# Autodesk Inventor assembly: GFRP_T2_06
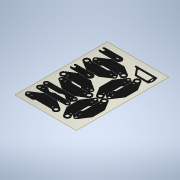
[picture p0: Inventor's stored thumbnail of the model, 180x180]
Saved by Autodesk Inventor 2020 (Build 240168000, 168)
## iProperties
Created: 2021-08-27
Part Number: GFRP_T2_06
Document SubType Name: Assembly
Designer: Masato
Author: Masato
## Documents named in this file (6)
- C:\Users\naoki\Documents\Inventor\CitBrains\git_clone\SUSTAINA_ver1_0\A_T2_175\SUSTAINA-OP\Cam\GFRP_T2_06.iam
- C:\Users\naoki\Documents\Inventor\CitBrains\git_clone\SUSTAINA_ver1_0\A_T2_175\SUSTAINA-OP\Cam\DisposableBoard.ipt
- C:\Users\naoki\Documents\Inventor\CitBrains\git_clone\SUSTAINA_ver1_0\A_T2_175\SUSTAINA-OP\LowerBody\Link\BackLink_frame.ipt
- C:\Users\naoki\Documents\Inventor\CitBrains\git_clone\SUSTAINA_ver1_0\A_T2_175\SUSTAINA-OP\LowerBody\Link\FrontLink_frame.ipt
- C:\Users\naoki\Documents\Inventor\CitBrains\git_clone\SUSTAINA_ver1_0\A_T2_175\SUSTAINA-OP\UpperBody\Arm\UpperArm_side_frame.ipt
- C:\Users\naoki\Documents\Inventor\CitBrains\git_clone\SUSTAINA_ver1_0\A_T2_175\SUSTAINA-OP\UpperBody\Arm\ForeArm_inside_frame.ipt
## Components (15 placed, 5 different names)
1. DisposableBoard:1 — メイト:2, メイト:1, フラッシュ:1, フラッシュ:2, メイト:4, メイト:5, 正接:1, 正接:2, メイト:9, 正接:5, メイト:18, メイト:19, 角度:2, 角度:3, 角度:4, メイト:25, メイト:26, メイト:31, 正接:16, 角度:5, メイト:32, メイト:33, 角度:6, メイト:34, フラッシュ:3, 正接:18, 正接:20, メイト:40, 正接:21, メイト:41, 角度:8, 正接:23, メイト:43, フラッシュ:4
2. FrontLink_frame:2 — メイト:9, 正接:5, 正接:7, メイト:17, 正接:17, 正接:22
3. FrontLink_frame:6 — メイト:16, メイト:18, 正接:12, 正接:13, 正接:22
4. FrontLink_frame:7 — メイト:16, メイト:19, 角度:4, 正接:13, 正接:24
5. FrontLink_frame:8 — メイト:17, 角度:3, メイト:31, 正接:12, 正接:17
6. BackLink_frame:2 — メイト:5, メイト:6, 正接:1, 角度:2, メイト:35
7. BackLink_frame:1 — メイト:4, メイト:6, 正接:2, 正接:7, メイト:20
8. FrontLink_frame:9 — メイト:20, メイト:23, メイト:25, 正接:15
9. FrontLink_frame:10 — メイト:23, メイト:26, 正接:15, 正接:16, メイト:36, メイト:39
10. FrontLink_frame:13 — 角度:5, メイト:34, フラッシュ:3, 正接:18, メイト:35
11. UpperArm_side_frame:3 — メイト:41, 角度:8, 正接:24, フラッシュ:4
12. FrontLink_frame:14 — メイト:32, 角度:6, 角度:7, メイト:38, 正接:19, メイト:42
13. FrontLink_frame:15 — メイト:33, 角度:7, メイト:37, メイト:38, 正接:19, 正接:20
14. ForeArm_inside_frame:1 — メイト:36, メイト:37, メイト:39, メイト:40, 正接:21
15. ForeArm_inside_frame:2 — メイト:42, 正接:23, メイト:43
## Relationships (54: Mate 27, Tangent 16, Angle 7, Flush 4)
- メイト:2 [Mate]: DisposableBoard:1
- メイト:1 [Mate]: DisposableBoard:1
- フラッシュ:1 [Flush]: DisposableBoard:1
- フラッシュ:2 [Flush]: DisposableBoard:1
- メイト:4 [Mate]: DisposableBoard:1 ↔ BackLink_frame:1
- メイト:5 [Mate]: DisposableBoard:1 ↔ BackLink_frame:2
- メイト:6 [Mate] (2.5 mm): BackLink_frame:2 ↔ BackLink_frame:1
- 正接:1 [Tangent] (2 mm): DisposableBoard:1 ↔ BackLink_frame:2
- 正接:2 [Tangent] (2 mm): DisposableBoard:1 ↔ BackLink_frame:1
- メイト:9 [Mate]: DisposableBoard:1 ↔ FrontLink_frame:2
- 正接:5 [Tangent] (2.5 mm): DisposableBoard:1 ↔ FrontLink_frame:2
- 正接:7 [Tangent] (2.5 mm): FrontLink_frame:2 ↔ BackLink_frame:1
- メイト:16 [Mate] (2.5 mm): FrontLink_frame:6 ↔ FrontLink_frame:7
- メイト:17 [Mate] (2.5 mm): FrontLink_frame:2 ↔ FrontLink_frame:8
- メイト:18 [Mate]: DisposableBoard:1 ↔ FrontLink_frame:6
- メイト:19 [Mate]: DisposableBoard:1 ↔ FrontLink_frame:7
- 角度:2 [Angle] (0 deg): DisposableBoard:1 ↔ BackLink_frame:2
- 角度:3 [Angle] (0 deg): DisposableBoard:1 ↔ FrontLink_frame:8
- 角度:4 [Angle] (0 deg): DisposableBoard:1 ↔ FrontLink_frame:7
- メイト:20 [Mate] (2.5 mm): BackLink_frame:1 ↔ FrontLink_frame:9
- メイト:23 [Mate] (2.5 mm): FrontLink_frame:9 ↔ FrontLink_frame:10
- メイト:25 [Mate]: DisposableBoard:1 ↔ FrontLink_frame:9
- メイト:26 [Mate]: DisposableBoard:1 ↔ FrontLink_frame:10
- メイト:31 [Mate]: DisposableBoard:1 ↔ FrontLink_frame:8
- 正接:12 [Tangent] (2.5 mm): FrontLink_frame:6 ↔ FrontLink_frame:8
- 正接:13 [Tangent] (3 mm): FrontLink_frame:6 ↔ FrontLink_frame:7
- 正接:15 [Tangent] (3 mm): FrontLink_frame:9 ↔ FrontLink_frame:10
- 正接:16 [Tangent] (2 mm): DisposableBoard:1 ↔ FrontLink_frame:10
- 正接:17 [Tangent] (3 mm): FrontLink_frame:2 ↔ FrontLink_frame:8
- 角度:5 [Angle] (0 deg): DisposableBoard:1 ↔ FrontLink_frame:13
- メイト:32 [Mate]: DisposableBoard:1 ↔ FrontLink_frame:14
- メイト:33 [Mate]: DisposableBoard:1 ↔ FrontLink_frame:15
- 角度:6 [Angle] (0 deg): DisposableBoard:1 ↔ FrontLink_frame:14
- 角度:7 [Angle] (0 deg): FrontLink_frame:14 ↔ FrontLink_frame:15
- メイト:34 [Mate]: DisposableBoard:1 ↔ FrontLink_frame:13
- フラッシュ:3 [Flush] (2 mm): DisposableBoard:1 ↔ FrontLink_frame:13
- 正接:18 [Tangent] (2 mm): DisposableBoard:1 ↔ FrontLink_frame:13
- メイト:35 [Mate] (2.5 mm): BackLink_frame:2 ↔ FrontLink_frame:13
- メイト:36 [Mate] (2.5 mm): FrontLink_frame:10 ↔ ForeArm_inside_frame:1
- メイト:37 [Mate] (2.5 mm): FrontLink_frame:15 ↔ ForeArm_inside_frame:1
- メイト:38 [Mate] (2.5 mm): FrontLink_frame:14 ↔ FrontLink_frame:15
- 正接:19 [Tangent] (3 mm): FrontLink_frame:14 ↔ FrontLink_frame:15
- 正接:20 [Tangent] (2 mm): DisposableBoard:1 ↔ FrontLink_frame:15
- メイト:39 [Mate] (2.5 mm): FrontLink_frame:10 ↔ ForeArm_inside_frame:1
- メイト:40 [Mate]: DisposableBoard:1 ↔ ForeArm_inside_frame:1
- 正接:21 [Tangent] (2 mm): DisposableBoard:1 ↔ ForeArm_inside_frame:1
- 正接:22 [Tangent] (2.5 mm): FrontLink_frame:2 ↔ FrontLink_frame:6
- メイト:41 [Mate]: DisposableBoard:1 ↔ UpperArm_side_frame:3
- 角度:8 [Angle] (0 deg): DisposableBoard:1 ↔ UpperArm_side_frame:3
- メイト:42 [Mate] (2.5 mm): FrontLink_frame:14 ↔ ForeArm_inside_frame:2
- 正接:23 [Tangent] (2 mm): DisposableBoard:1 ↔ ForeArm_inside_frame:2
- メイト:43 [Mate]: DisposableBoard:1 ↔ ForeArm_inside_frame:2
- 正接:24 [Tangent] (2.5 mm): FrontLink_frame:7 ↔ UpperArm_side_frame:3
- フラッシュ:4 [Flush] (4 mm): DisposableBoard:1 ↔ UpperArm_side_frame:3
